# Autodesk Inventor assembly: Montagem_Arduino2
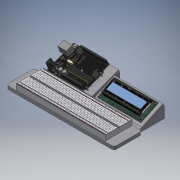
[picture p0: Inventor's stored thumbnail of the model, 180x180]
Saved by Autodesk Inventor 2017 (Build 210142000, 142)
## iProperties
Created: 2019-04-20
Part Number: Montagem_Arduino2
Description: MONTAGEM TRABALHO
Document SubType Name: Assembly
Designer: Marcus
Author: Marcus
CONJUNTO: TEXTO CONJUNTO
EQUIPAMENTO: TEXTO EQUIPAMENTO
SUBCONJUNTO: TEXTO SUBCONJUNTO
## Documents named in this file (5)
- C:\Users\Marcus\Google Drive\Metal Class Projetos\Base Arduino\Montagem_Arduino2.iam
- C:\Users\Marcus\Google Drive\Metal Class Projetos\Base Arduino\Plataforma2.ipt
- C:\Users\Marcus\Google Drive\Metal Class Projetos\Base Arduino\ArduinoUNO .ipt
- C:\Users\Marcus\Google Drive\Metal Class Projetos\Base Arduino\LCD.ipt
- C:\Users\Marcus\Google Drive\Metal Class Projetos\Base Arduino\Protoboard.ipt
## Components (4 placed, 4 different names)
1. Plataforma2:1 — Flush:1, Flush:2, Flush:3, Insert:1, Mate:1, Insert:2, Mate:2, Mate:3, Flush:4
2. ArduinoUNO :1 — Insert:1, Mate:1
3. LCD:1 — Insert:2, Mate:2
4. Protoboard:1 — Mate:3, Flush:4, Flush:5
## Relationships (10: Flush 5, Mate 3, Insert 2)
- Flush:1: Plataforma2:1
- Flush:2: Plataforma2:1
- Flush:3: Plataforma2:1
- Insert:1 (5 mm): Plataforma2:1 ↔ ArduinoUNO :1
- Mate:1: Plataforma2:1 ↔ ArduinoUNO :1
- Insert:2 (2 mm): Plataforma2:1 ↔ LCD:1
- Mate:2: Plataforma2:1 ↔ LCD:1
- Mate:3: Plataforma2:1 ↔ Protoboard:1
- Flush:4 (1 mm): Plataforma2:1 ↔ Protoboard:1
- Flush:5: Protoboard:1
